# Autodesk Inventor assembly: Remote Top Print Assembly
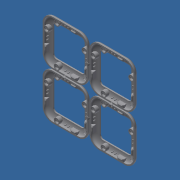
[picture p0: Inventor's stored thumbnail of the model, 180x180]
Saved by Autodesk Inventor 2,016 (Build 200138000, 138)
## iProperties
Created: 2015-10-14
Part Number: Remote Top Print Assembly
Document SubType Name: Assembly
Designer: Sam Clay
Author: Sam Clay
## Documents named in this file (2)
- Z:\enclosure\inventor\Remote Top Print Assembly.iam
- Z:\enclosure\inventor\Remote Top.ipt
## Components (4 placed, 1 different names)
1. Remote Top:1
2. Remote Top:2
3. Remote Top:3
4. Remote Top:4
## Component patterns: (4 elements, first: Remote Top:1)
